# Autodesk Inventor assembly: Pillars_18650_Assembly
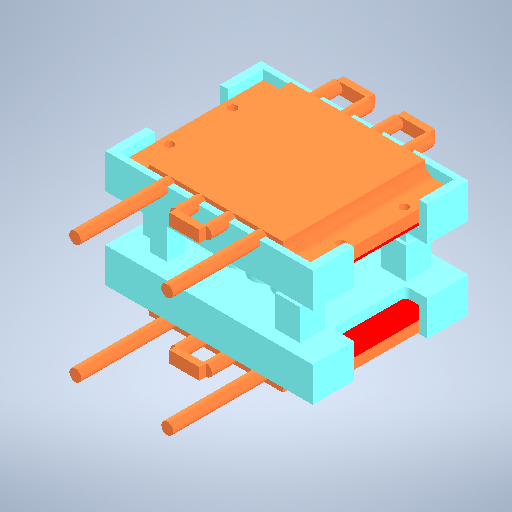
[picture p0: Inventor's stored thumbnail of the model, 512x512]
Saved by Autodesk Inventor 2025.2 (Build 292293000, 293)
## iProperties
Created: 2025-08-10
Part Number: Pillars_18650_Assembly
Document SubType Name: Assembly
Designer: cbast
Author: cbast
## Documents named in this file (5)
- C:\Users\cbast\OneDrive\Documents\Pillars_18650_Assembly.iam
- C:\Users\cbast\OneDrive\Documents\GitHub\Smart-Pack-for-Advanced-Research-and-Control\variations\Camden\V0.1\18650(PINK).ipt
- C:\Users\cbast\OneDrive\Documents\GitHub\Smart-Pack-for-Advanced-Research-and-Control\variations\Camden\V0.2\PILLARSCELLCASE18650.ipt
- C:\Users\cbast\OneDrive\Documents\GitHub\Smart-Pack-for-Advanced-Research-and-Control\variations\Camden\V0.1\thermal pad.ipt
- C:\Users\cbast\OneDrive\Documents\GitHub\Smart-Pack-for-Advanced-Research-and-Control\variations\Camden\V0.1\cooling plate.ipt
## Components (16 placed, 4 different names)
1. 18650(PINK):1 — Mate:5, Flush:2, Mate:14, Mate:15
2. 18650(PINK):2 — Mate:4, Flush:4
3. 18650(PINK):3 — Mate:6, Flush:5
4. 18650(PINK):4 — Mate:3, Flush:3
5. 18650(PINK):5 — Mate:2, Flush:1
6. 18650(PINK):6 — Mate:1, Flush:1, Flush:2, Flush:3, Flush:4, Flush:5, Flush:6, Flush:7, Flush:8, Flush:9, Mate:12
7. 18650(PINK):7 — Mate:7, Flush:6, Mate:13
8. 18650(PINK):8 — Mate:8, Flush:7
9. 18650(PINK):9 — Mate:9, Flush:8
10. 18650(PINK):10 — Mate:10, Flush:9
11. PILLARSCELLCASE18650:1 — Mate:1, Mate:2, Mate:3, Mate:4, Mate:5, Mate:6, Mate:7, Mate:8, Mate:9, Mate:10, Mate:11, Mate:18, Mate:19
12. PILLARSCELLCASE18650:2 — Mate:11, Mate:12, Mate:13, Mate:16, Mate:17, Mate:21, Mate:22
13. thermal pad:1 — Mate:14, Mate:18, Mate:19, Mate:25
14. thermal pad:2 — Mate:15, Mate:16, Mate:17, Mate:20
15. cooling plate:1 — Mate:20, Mate:21, Mate:22, Mate:23, Mate:24
16. cooling plate:2 — Mate:23, Mate:24, Mate:25
## Relationships (34: Mate 25, Flush 9)
- Mate:1: 18650(PINK):6 ↔ PILLARSCELLCASE18650:1
- Mate:2: 18650(PINK):5 ↔ PILLARSCELLCASE18650:1
- Mate:3: 18650(PINK):4 ↔ PILLARSCELLCASE18650:1
- Mate:4: 18650(PINK):2 ↔ PILLARSCELLCASE18650:1
- Mate:5: 18650(PINK):1 ↔ PILLARSCELLCASE18650:1
- Mate:6: 18650(PINK):3 ↔ PILLARSCELLCASE18650:1
- Mate:7: 18650(PINK):7 ↔ PILLARSCELLCASE18650:1
- Mate:8: 18650(PINK):8 ↔ PILLARSCELLCASE18650:1
- Mate:9: 18650(PINK):9 ↔ PILLARSCELLCASE18650:1
- Mate:10: 18650(PINK):10 ↔ PILLARSCELLCASE18650:1
- Mate:11: PILLARSCELLCASE18650:1 ↔ PILLARSCELLCASE18650:2
- Flush:1: 18650(PINK):5 ↔ 18650(PINK):6
- Flush:2: 18650(PINK):1 ↔ 18650(PINK):6
- Flush:3: 18650(PINK):4 ↔ 18650(PINK):6
- Flush:4: 18650(PINK):2 ↔ 18650(PINK):6
- Flush:5: 18650(PINK):3 ↔ 18650(PINK):6
- Flush:6: 18650(PINK):6 ↔ 18650(PINK):7
- Flush:7: 18650(PINK):6 ↔ 18650(PINK):8
- Flush:8: 18650(PINK):6 ↔ 18650(PINK):9
- Flush:9: 18650(PINK):6 ↔ 18650(PINK):10
- Mate:12: 18650(PINK):6 ↔ PILLARSCELLCASE18650:2
- Mate:13: 18650(PINK):7 ↔ PILLARSCELLCASE18650:2
- Mate:14: 18650(PINK):1 ↔ thermal pad:1
- Mate:15: 18650(PINK):1 ↔ thermal pad:2
- Mate:16: PILLARSCELLCASE18650:2 ↔ thermal pad:2
- Mate:17: PILLARSCELLCASE18650:2 ↔ thermal pad:2
- Mate:18: PILLARSCELLCASE18650:1 ↔ thermal pad:1
- Mate:19: PILLARSCELLCASE18650:1 ↔ thermal pad:1
- Mate:20: thermal pad:2 ↔ cooling plate:1
- Mate:21: PILLARSCELLCASE18650:2 ↔ cooling plate:1
- Mate:22: PILLARSCELLCASE18650:2 ↔ cooling plate:1
- Mate:23: cooling plate:1 ↔ cooling plate:2
- Mate:24: cooling plate:1 ↔ cooling plate:2
- Mate:25: thermal pad:1 ↔ cooling plate:2
